# Autodesk Inventor assembly: Rahmen
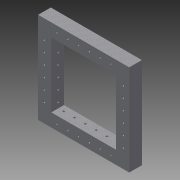
[picture p0: Inventor's stored thumbnail of the model, 180x180]
Saved by Autodesk Inventor 2015 (Build 190159000, 159)
## iProperties
Created: 2016-04-07
Part Number: Rahmen
Document SubType Name: Assembly
Designer: Carl
Author: Carl
## Documents named in this file (2)
- D:\Eigene Dateien\Dokumente\Uni\Master\Sketching with Hardware\swh2016\Rahmen.iam
- D:\Eigene Dateien\Dokumente\Uni\Master\Sketching with Hardware\swh2016\Platte6mm.ipt
## Components (8 placed, 1 different names)
1. Platte6mm:1 — Passend:1, Fluchtend:3, Fluchtend:11, Passend:4
2. Platte6mm:2 — Passend:1, Fluchtend:4, Fluchtend:10, Passend:5
3. Platte6mm:3 — Fluchtend:5, Fluchtend:9, Passend:5, Passend:6
4. Platte6mm:4 — Fluchtend:6, Fluchtend:8, Passend:6, Passend:7
5. Platte6mm:5 — Fluchtend:7, Fluchtend:8, Fluchtend:9, Fluchtend:10, Fluchtend:11, Fluchtend:12, Fluchtend:13, Fluchtend:14, Passend:7
6. Platte6mm:6 — Fluchtend:2, Fluchtend:12, Passend:3, Passend:4
7. Platte6mm:7 — Fluchtend:1, Fluchtend:2, Fluchtend:3, Fluchtend:4, Fluchtend:5, Fluchtend:6, Fluchtend:7, Fluchtend:14, Passend:2
8. Platte6mm:8 — Fluchtend:1, Fluchtend:13, Passend:2, Passend:3
## Relationships (21: Flush 14, Mate 7)
- Passend:1 [Mate]: Platte6mm:1 ↔ Platte6mm:2
- Fluchtend:1 [Flush]: Platte6mm:7 ↔ Platte6mm:8
- Fluchtend:2 [Flush]: Platte6mm:6 ↔ Platte6mm:7
- Fluchtend:3 [Flush]: Platte6mm:1 ↔ Platte6mm:7
- Fluchtend:4 [Flush]: Platte6mm:2 ↔ Platte6mm:7
- Fluchtend:5 [Flush]: Platte6mm:3 ↔ Platte6mm:7
- Fluchtend:6 [Flush]: Platte6mm:4 ↔ Platte6mm:7
- Fluchtend:7 [Flush]: Platte6mm:5 ↔ Platte6mm:7
- Fluchtend:8 [Flush]: Platte6mm:4 ↔ Platte6mm:5
- Fluchtend:9 [Flush]: Platte6mm:3 ↔ Platte6mm:5
- Fluchtend:10 [Flush]: Platte6mm:2 ↔ Platte6mm:5
- Fluchtend:11 [Flush]: Platte6mm:1 ↔ Platte6mm:5
- Fluchtend:12 [Flush]: Platte6mm:5 ↔ Platte6mm:6
- Fluchtend:13 [Flush]: Platte6mm:5 ↔ Platte6mm:8
- Fluchtend:14 [Flush]: Platte6mm:5 ↔ Platte6mm:7
- Passend:2 [Mate]: Platte6mm:7 ↔ Platte6mm:8
- Passend:3 [Mate]: Platte6mm:6 ↔ Platte6mm:8
- Passend:4 [Mate]: Platte6mm:1 ↔ Platte6mm:6
- Passend:5 [Mate]: Platte6mm:2 ↔ Platte6mm:3
- Passend:6 [Mate]: Platte6mm:3 ↔ Platte6mm:4
- Passend:7 [Mate]: Platte6mm:4 ↔ Platte6mm:5
